# Autodesk Inventor assembly: Lady Brown
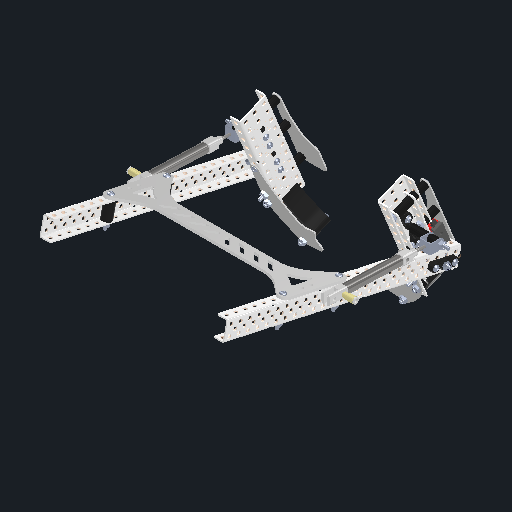
[picture p0: Inventor's stored thumbnail of the model, 512x512]
Saved by Autodesk Inventor 2025.1 (Build 291241000, 241)
## iProperties
Created: 2024-12-19
Part Number: Lady Brown
Document SubType Name: Assembly
Designer: Juan
Author: Juan
## Documents named in this file (36)
- C:\Users\Juanl\Documents\GitHub\ATUM-V5RC-High-Stakes-CAD\Robot\Subassemblies\Lady Brown.iam
- C:\Users\Juanl\Documents\GitHub\ATUM-V5RC-High-Stakes-CAD\VEX-CAD-Inventor\Structure\C Channel\Aluminum 1x2x1\Alu C 1x2x1x25.ipt
- C:\Users\Juanl\Documents\GitHub\ATUM-V5RC-High-Stakes-CAD\VEX-CAD-Inventor\Motion\Spacers\Spacer Nylon .375 OD\NSpacer .375 OD x .500.ipt
- C:\Users\Juan\Documents\GitHub\ATUM-VRC-High-Stakes-CAD\VEX-CAD-Inventor\Motion\Spacers\Spacer Nylon .375 OD.ipt
- C:\Users\Juanl\Documents\GitHub\ATUM-V5RC-High-Stakes-CAD\VEX-CAD-Inventor\Motion\Pneumatics\Reference Parts\Pistons\Double Acting Piston Body.ipt
- C:\Users\Juanl\Documents\GitHub\ATUM-V5RC-High-Stakes-CAD\VEX-CAD-Inventor\Motion\Pneumatics\Reference Parts\Pistons\Double Acting Piston Rod.ipt
- C:\Users\Juanl\Documents\GitHub\ATUM-V5RC-High-Stakes-CAD\VEX-CAD-Inventor\Motion\Pneumatics\Legacy - SMC Pneumatics\Fitting for Cylinders.ipt
- C:\Users\Juanl\Documents\GitHub\ATUM-V5RC-High-Stakes-CAD\VEX-CAD-Inventor\Motion\Shaft LS\Bearing Flat.ipt
- C:\Users\Juanl\Documents\GitHub\ATUM-V5RC-High-Stakes-CAD\VEX-CAD-Inventor\Structure\Hardware\Screw Steel - Star\SScrew Star Smooth .500.ipt
- C:\Users\Juan\Documents\GitHub\ATUM-VRC-High-Stakes-CAD\VEX-CAD-Inventor\Structure\Hardware\Screw Steel - Star.ipt
- C:\Users\Juanl\Documents\GitHub\ATUM-V5RC-High-Stakes-CAD\VEX-CAD-Inventor\Structure\C Channel\Aluminum 1x3x1\Alu C 1x3x1x11.ipt
- C:\Users\Juanl\Documents\GitHub\ATUM-V5RC-High-Stakes-CAD\VEX-CAD-Inventor\Motion\1-Post Bearing Flat Hex Retainer.ipt
- C:\Users\Juanl\Documents\GitHub\ATUM-V5RC-High-Stakes-CAD\VEX-CAD-Inventor\Motion\Pneumatics\Legacy - SMC Pneumatics\Cylinder Mount.ipt
- C:\Users\Juanl\Documents\GitHub\ATUM-V5RC-High-Stakes-CAD\VEX-CAD-Inventor\Motion\Spacers\Spacer Nylon .375 OD\NSpacer .375 OD x .375.ipt
- C:\Users\Juanl\Documents\GitHub\ATUM-V5RC-High-Stakes-CAD\VEX-CAD-Inventor\Structure\Hardware\Screw Steel - Star\SScrew Star Smooth 2.250.ipt
- C:\Users\Juanl\Documents\GitHub\ATUM-V5RC-High-Stakes-CAD\VEX-CAD-Inventor\Structure\Hardware\Nut Nylock.ipt
- C:\Users\Juanl\Documents\GitHub\ATUM-V5RC-High-Stakes-CAD\VEX-CAD-Inventor\Structure\Hardware\Screw Steel - Star\SScrew Star Smooth 1.750.ipt
- C:\Users\Juanl\Documents\GitHub\ATUM-V5RC-High-Stakes-CAD\VEX-CAD-Inventor\Structure\Hardware\Nut Thin Nylock.ipt
- C:\Users\Juanl\Documents\GitHub\ATUM-V5RC-High-Stakes-CAD\VEX-CAD-Inventor\Structure\Hardware\Screw Steel - Star\SScrew Star Smooth .375.ipt
- C:\Users\Juanl\Documents\GitHub\ATUM-V5RC-High-Stakes-CAD\VEX-CAD-Inventor\Motion\Spacers\Spacer Nylon .375 OD\NSpacer .375 OD x .250.ipt
- C:\Users\Juanl\Documents\GitHub\ATUM-V5RC-High-Stakes-CAD\Protobot\Lady Brown Tabs.ipt
- C:\Users\Juanl\Documents\GitHub\ATUM-V5RC-High-Stakes-CAD\Protobot\Lady Brown Tab Top.ipt
- C:\Users\Juanl\Documents\GitHub\ATUM-V5RC-High-Stakes-CAD\VEX-CAD-Inventor\Structure\C Channel\Aluminum 1x2x1\Alu C 1x2x1x8.ipt
- C:\Users\Juanl\Documents\GitHub\ATUM-V5RC-High-Stakes-CAD\VEX-CAD-Inventor\Electronics\Sensors\Line Tracker - V2.ipt
- C:\Users\Juanl\Documents\GitHub\ATUM-V5RC-High-Stakes-CAD\Protobot\Lady Brown Ring Stop.ipt
- C:\Users\Juanl\Documents\GitHub\ATUM-V5RC-High-Stakes-CAD\VEX-CAD-Inventor\Motion\Spacers\Washer Steel\SWasher .375 OD x .062500.ipt
- C:\Users\Juan\Documents\GitHub\ATUM-VRC-High-Stakes-CAD\VEX-CAD-Inventor\Motion\Spacers\Washer Steel.ipt
- C:\Users\Juanl\Documents\GitHub\ATUM-V5RC-High-Stakes-CAD\VEX-CAD-Inventor\Structure\Hardware\Screw Steel - Star\SScrew Star Smooth 1.500.ipt
- C:\Users\Juanl\Documents\GitHub\ATUM-V5RC-High-Stakes-CAD\VEX-CAD-Inventor\Structure\Hardware\Screw Steel - Star\SScrew Star Smooth 2.000.ipt
- C:\Users\Juanl\Documents\GitHub\ATUM-V5RC-High-Stakes-CAD\VEX-CAD-Inventor\Structure\Hardware\Screw Steel - Star\SScrew Star Smooth 2.500.ipt
- C:\Users\Juanl\Documents\GitHub\ATUM-V5RC-High-Stakes-CAD\VEX-CAD-Inventor\Structure\Hardware\Screw Steel - Star\SScrew Star Smooth 1.250.ipt
- C:\Users\Juanl\Documents\GitHub\ATUM-V5RC-High-Stakes-CAD\VEX-CAD-Inventor\Structure\Hardware\Screw Steel - Star\SScrew Star Smooth .625.ipt
- C:\Users\Juanl\Documents\GitHub\ATUM-V5RC-High-Stakes-CAD\Protobot\Lady Brown Arm Brace.ipt
- C:\Users\Juanl\Documents\GitHub\ATUM-V5RC-High-Stakes-CAD\VEX-CAD-Inventor\Motion\Spacers\Spacer Nylon .500 OD\NSpacer Black .500 OD x .500.ipt
- C:\Users\Juan\Documents\GitHub\ATUM-VRC-High-Stakes-CAD\VEX-CAD-Inventor\Motion\Spacers\Spacer Nylon .500 OD.ipt
- C:\Users\Juanl\Documents\GitHub\ATUM-V5RC-High-Stakes-CAD\VEX-CAD-Inventor\Motion\Spacers\Spacer Nylon .500 OD\NSpacer Black .500 OD x .375.ipt
## Components (130 placed, 31 different names)
1. Alu C 1x2x1x25:1 — Mate:103, Mate:104, Mate:105, Rigid:86, Rigid:91, Rigid:98, Rigid:99
2. Alu C 1x2x1x25:2 — Rigid:92, Rigid:93, Rigid:96, Rigid:97
3. Double Acting Piston Body:1
4. Double Acting Piston Rod:1
5. Fitting for Cylinders:1
6. Bearing Flat:1
7. SScrew Star Smooth .500:1
8. SScrew Star Smooth .500:2
9. Alu C 1x3x1x11:1
10. 1-Post Bearing Flat Hex Retainer:1
11. 1-Post Bearing Flat Hex Retainer:2 — Mate:77
12. Cylinder Mount:1
13. NSpacer .375 OD x .375:3 — Mate:78
14. NSpacer .375 OD x .500:4 — Mate:79
15. NSpacer .375 OD x .375:5
16. NSpacer .375 OD x .500:6
17. SScrew Star Smooth 2.250:3
18. Nut Nylock:1
19. SScrew Star Smooth 1.750:4
20. Nut Thin Nylock:1
21. Nut Nylock:2
22. SScrew Star Smooth .375:5
23. SScrew Star Smooth .375:6
24. Nut Nylock:3
25. Double Acting Piston Body:2
26. Double Acting Piston Rod:2
27. NSpacer .375 OD x .500:13
28. NSpacer .375 OD x .375:14
29. Nut Thin Nylock:4
30. Nut Thin Nylock:3
31. Nut Thin Nylock:6
32. Nut Thin Nylock:5
33. SScrew Star Smooth 2.250:12
34. NSpacer .375 OD x .500:12
35. Fitting for Cylinders:2
36. Bearing Flat:2
37. SScrew Star Smooth .500:7
38. SScrew Star Smooth .500:8
39. Alu C 1x3x1x11:2
40. Cylinder Mount:2
41. NSpacer .375 OD x .500:7
42. Nut Nylock:4
43. Nut Thin Nylock:2
44. Nut Nylock:5
45. SScrew Star Smooth .375:9
46. SScrew Star Smooth .375:10
47. Nut Nylock:6
48. 1-Post Bearing Flat Hex Retainer:3 — Mate:93
49. 1-Post Bearing Flat Hex Retainer:4 — Mate:94
50. SScrew Star Smooth 1.750:11
51. NSpacer .375 OD x .500:8 — Mate:95
52. NSpacer .375 OD x .375:9
53. NSpacer .375 OD x .375:15 — Rigid:36, Rigid:41
54. NSpacer .375 OD x .375:16 — Rigid:36, Mate:73, Mate:75, Mate:76
55. NSpacer .375 OD x .250:17 — Mate:70, Mate:72, Rigid:42
56. NSpacer .375 OD x .250:18 — Mate:71, Rigid:43
57. Lady Brown Tabs:2 — Mate:70, Mate:71, Mate:72, Mate:88, Rigid:54, Rigid:56, Rigid:67, Rigid:68, Rigid:78, Rigid:83
58. Lady Brown Tab Top:1 — Mate:73, Mate:75, Mate:76, Mate:83, Rigid:72, Rigid:76, Rigid:79
59. NSpacer .375 OD x .375:21 — Rigid:40
60. NSpacer .375 OD x .375:22 — Mate:83
61. Alu C 1x2x1x8:1 — Mate:77, Mate:78, Mate:79, Rigid:40, Rigid:41, Rigid:42, Rigid:43, Flush:1, Mate:84, Mate:85, Rigid:45, Mate:86, Mate:87, Rigid:71, Rigid:74, Rigid:81, Rigid:84
62. Line Tracker - V2:2 — Flush:1, Mate:84, Mate:85
63. NSpacer .375 OD x .375:23 — Rigid:45
64. NSpacer .375 OD x .375:24
65. Lady Brown Ring Stop:1 — Mate:86, Mate:87, Mate:88, Rigid:62, Rigid:63
66. Lady Brown Ring Stop:2 — Mate:97, Mate:98, Mate:102, Rigid:64, Rotational:3
67. Lady Brown Tabs:3 — Mate:92, Mate:96, Mate:102, Rigid:53, Rigid:55, Rigid:65, Rigid:66, Rigid:77, Rotational:5
68. NSpacer .375 OD x .250:25 — Rigid:46
69. NSpacer .375 OD x .250:26 — Mate:92, Rigid:47, Mate:96
70. Lady Brown Tab Top:2 — Mate:99, Mate:100, Mate:101, Rigid:73, Rigid:75, Rigid:80
71. Alu C 1x2x1x8:2 — Mate:93, Mate:94, Mate:95, Rigid:46, Rigid:47, Mate:97, Mate:98, Mate:99, Mate:100, Rigid:51, Rigid:52, Rotational:2, Rigid:61, Rotational:4, Rigid:82, Rigid:85
72. NSpacer .375 OD x .375:27 — Rigid:51
73. NSpacer .375 OD x .375:28
74. NSpacer .375 OD x .375:29 — Rigid:52
75. NSpacer .375 OD x .375:30 — Mate:101
76. NSpacer .375 OD x .375:31 — Rotational:2
77. NSpacer .375 OD x .375:32
78. NSpacer .375 OD x .250:33 — Rigid:54, Rigid:57
79. NSpacer .375 OD x .250:34 — Rigid:53, Rigid:60
80. NSpacer .375 OD x .250:35 — Rigid:56, Rigid:58
81. NSpacer .375 OD x .250:36 — Rigid:55, Rigid:59
82. SWasher .375 OD x .062500:1 — Rigid:58
83. SWasher .375 OD x .062500:2 — Rigid:57
84. SWasher .375 OD x .062500:3 — Rigid:60
85. SWasher .375 OD x .062500:4 — Rigid:59
86. NSpacer .375 OD x .375:37 — Rigid:61, Rigid:69
87. SScrew Star Smooth 1.500:13 — Rotational:3
88. SScrew Star Smooth 1.500:14 — Rigid:64
89. SScrew Star Smooth 1.500:15 — Rigid:63
90. SScrew Star Smooth 1.500:16 — Rigid:62
91. Nut Thin Nylock:7 — Rigid:65
92. Nut Thin Nylock:8 — Rigid:66
93. Nut Thin Nylock:9 — Rigid:68
94. Nut Thin Nylock:10 — Rigid:67
95. NSpacer .375 OD x .500:38 — Rigid:69
96. NSpacer .375 OD x .375:39 — Rigid:71
97. NSpacer .375 OD x .500:40
98. SScrew Star Smooth 2.000:17 — Rigid:72
99. SScrew Star Smooth 2.000:18 — Rigid:73
100. Nut Thin Nylock:11 — Rigid:74
101. Nut Thin Nylock:12 — Rotational:4
102. SScrew Star Smooth 2.500:20 — Rigid:75
103. SScrew Star Smooth 2.500:21 — Rigid:76
104. Nut Thin Nylock:13 — Rigid:78
105. Nut Thin Nylock:14 — Rigid:77
106. SScrew Star Smooth 1.250:22 — Rigid:80
107. SScrew Star Smooth 1.250:23 — Rigid:79
108. Nut Thin Nylock:15 — Rigid:82
109. Nut Thin Nylock:16 — Rigid:81
110. SScrew Star Smooth .625:24 — Rotational:5
111. SScrew Star Smooth .625:25 — Rigid:83
112. Nut Thin Nylock:17 — Rigid:85
113. Nut Thin Nylock:18 — Rigid:84
114. Lady Brown Arm Brace:1 — Mate:103, Mate:104, Mate:105, Rotational:6, Rigid:94, Rigid:95, Rotational:7
115. NSpacer Black .500 OD x .500:1 — Rigid:86, Rigid:87
116. NSpacer Black .500 OD x .375:2 — Rigid:87
117. NSpacer Black .500 OD x .500:3 — Rigid:91
118. NSpacer Black .500 OD x .375:4
119. NSpacer Black .500 OD x .500:5 — Rigid:93
120. NSpacer Black .500 OD x .375:6
121. NSpacer Black .500 OD x .500:7 — Rigid:92
122. NSpacer Black .500 OD x .375:8
123. SScrew Star Smooth 1.500:26 — Rigid:94
124. SScrew Star Smooth 1.500:27 — Rotational:6
125. SScrew Star Smooth 1.500:28 — Rotational:7
126. SScrew Star Smooth 1.500:29 — Rigid:95
127. Nut Nylock:7 — Rigid:97
128. Nut Nylock:8 — Rigid:96
129. Nut Nylock:9 — Rigid:98
130. Nut Nylock:10 — Rigid:99
## Relationships (177: WeldJoint 94, Mate 73, RevoluteJoint 7, CylindricalJoint 2, Flush 1)
- [Mate]: Double Acting Piston Body:1 ↔ Double Acting Piston Rod:1
- [CylindricalJoint]: Double Acting Piston Body:1 ↔ Double Acting Piston Rod:1
- [Mate]: Double Acting Piston Body:1 ↔ Fitting for Cylinders:1
- [Mate]: Double Acting Piston Body:1 ↔ Fitting for Cylinders:1
- [Mate]: Alu C 1x2x1x25:1 ↔ Bearing Flat:1
- [Mate]: Alu C 1x2x1x25:1 ↔ Bearing Flat:1
- [Mate]: Alu C 1x2x1x25:1 ↔ Bearing Flat:1
- [WeldJoint]: Bearing Flat:1 ↔ SScrew Star Smooth .500:2
- [WeldJoint]: Bearing Flat:1 ↔ SScrew Star Smooth .500:1
- [Mate]: Alu C 1x3x1x11:1 ↔ 1-Post Bearing Flat Hex Retainer:2
- [Mate]: Alu C 1x3x1x11:1 ↔ 1-Post Bearing Flat Hex Retainer:2
- [Mate]: Alu C 1x3x1x11:1 ↔ 1-Post Bearing Flat Hex Retainer:1
- [Mate]: Alu C 1x3x1x11:1 ↔ 1-Post Bearing Flat Hex Retainer:1
- [Mate]: Alu C 1x3x1x11:1 ↔ 1-Post Bearing Flat Hex Retainer:2
- [Mate]: Alu C 1x3x1x11:1 ↔ 1-Post Bearing Flat Hex Retainer:1
- [Mate]: Bearing Flat:1 ↔ 1-Post Bearing Flat Hex Retainer:2
- [Mate]: Double Acting Piston Rod:1 ↔ Cylinder Mount:1
- [Mate]: 1-Post Bearing Flat Hex Retainer:1 ↔ Cylinder Mount:1
- [WeldJoint]: NSpacer .375 OD x .500:4 ↔ NSpacer .375 OD x .375:5
- [Mate]: Cylinder Mount:1 ↔ NSpacer .375 OD x .500:6
- [Mate]: Cylinder Mount:1 ↔ NSpacer .375 OD x .500:6
- [WeldJoint]: Alu C 1x3x1x11:1 ↔ SScrew Star Smooth 2.250:3
- [WeldJoint]: Cylinder Mount:1 ↔ Nut Nylock:1
- [WeldJoint]: Alu C 1x3x1x11:1 ↔ SScrew Star Smooth 1.750:4
- [WeldJoint]: Bearing Flat:1 ↔ Nut Thin Nylock:1
- [WeldJoint]: Alu C 1x3x1x11:1 ↔ SScrew Star Smooth .375:6
- [WeldJoint]: Alu C 1x3x1x11:1 ↔ SScrew Star Smooth .375:5
- [WeldJoint]: 1-Post Bearing Flat Hex Retainer:1 ↔ Nut Nylock:2
- [WeldJoint]: 1-Post Bearing Flat Hex Retainer:2 ↔ Nut Nylock:3
- [Mate]: Double Acting Piston Body:2 ↔ Double Acting Piston Rod:2
- [Mate]: Double Acting Piston Body:2 ↔ Fitting for Cylinders:2
- [Mate]: Double Acting Piston Body:2 ↔ Fitting for Cylinders:2
- [Mate]: Double Acting Piston Rod:2 ↔ Cylinder Mount:2
- [Mate]: Cylinder Mount:2 ↔ NSpacer .375 OD x .500:7
- [CylindricalJoint]: Double Acting Piston Body:2 ↔ Double Acting Piston Rod:2
- [WeldJoint]: Bearing Flat:2 ↔ SScrew Star Smooth .500:7
- [WeldJoint]: Bearing Flat:2 ↔ SScrew Star Smooth .500:8
- [WeldJoint]: Cylinder Mount:2 ↔ Nut Nylock:4
- [WeldJoint]: Bearing Flat:2 ↔ Nut Thin Nylock:2
- [WeldJoint]: Alu C 1x3x1x11:2 ↔ SScrew Star Smooth .375:9
- [WeldJoint]: Alu C 1x3x1x11:2 ↔ SScrew Star Smooth .375:10
- [Mate]: Alu C 1x3x1x11:2 ↔ 1-Post Bearing Flat Hex Retainer:3
- [Mate]: Alu C 1x3x1x11:2 ↔ 1-Post Bearing Flat Hex Retainer:3
- [Mate]: Alu C 1x3x1x11:2 ↔ 1-Post Bearing Flat Hex Retainer:3
- [Mate]: Alu C 1x3x1x11:2 ↔ 1-Post Bearing Flat Hex Retainer:4
- [Mate]: Alu C 1x3x1x11:2 ↔ 1-Post Bearing Flat Hex Retainer:4
- [Mate]: Alu C 1x3x1x11:2 ↔ 1-Post Bearing Flat Hex Retainer:4
- [WeldJoint]: Alu C 1x3x1x11:2 ↔ SScrew Star Smooth 1.750:11
- [Mate]: Alu C 1x2x1x25:2 ↔ Bearing Flat:2
- [Mate]: Alu C 1x2x1x25:2 ↔ Bearing Flat:2
- [Mate]: Alu C 1x2x1x25:2 ↔ Bearing Flat:2
- [Mate]: Bearing Flat:2 ↔ SScrew Star Smooth 1.750:11
- [Mate]: Cylinder Mount:2 ↔ NSpacer .375 OD x .500:7
- [WeldJoint]: Nut Nylock:5 ↔ 1-Post Bearing Flat Hex Retainer:3
- [WeldJoint]: Nut Nylock:6 ↔ 1-Post Bearing Flat Hex Retainer:4
- [WeldJoint]: NSpacer .375 OD x .500:8 ↔ NSpacer .375 OD x .375:9
- [Mate]: Alu C 1x2x1x25:2 ↔ Double Acting Piston Body:2
- [Mate] (0.7937 mm): Alu C 1x2x1x25:2 ↔ Double Acting Piston Body:2
- [Mate]: Alu C 1x3x1x11:1 ↔ Alu C 1x3x1x11:2
- [Mate]: Alu C 1x3x1x11:1 ↔ Alu C 1x3x1x11:2
- [RevoluteJoint] (0.7937 mm): Alu C 1x2x1x25:1 ↔ Double Acting Piston Body:1
- [WeldJoint] (6.35 mm): Double Acting Piston Rod:1 ↔ Cylinder Mount:1
- [WeldJoint] (6.35 mm): Double Acting Piston Rod:2 ↔ Cylinder Mount:2
- [Mate]: Cylinder Mount:2 ↔ NSpacer .375 OD x .375:9
- [Mate]: 1-Post Bearing Flat Hex Retainer:2 ↔ NSpacer .375 OD x .375:3
- [WeldJoint]: Cylinder Mount:1 ↔ NSpacer .375 OD x .375:5
- [WeldJoint]: Alu C 1x2x1x25:1 ↔ NSpacer .375 OD x .500:12
- [WeldJoint]: NSpacer .375 OD x .375:3 ↔ NSpacer .375 OD x .500:12
- [WeldJoint]: NSpacer .375 OD x .500:13 ↔ NSpacer .375 OD x .375:14
- [Mate]: NSpacer .375 OD x .500:13 ↔ SScrew Star Smooth 1.750:11
- [Mate]: Alu C 1x2x1x25:2 ↔ NSpacer .375 OD x .500:13
- [Mate]: NSpacer .375 OD x .375:14 ↔ 1-Post Bearing Flat Hex Retainer:4
- [WeldJoint]: Alu C 1x2x1x25:1 ↔ Nut Thin Nylock:4
- [WeldJoint]: Alu C 1x2x1x25:1 ↔ Nut Thin Nylock:3
- [WeldJoint]: SScrew Star Smooth 2.250:12 ↔ Alu C 1x3x1x11:2
- [WeldJoint]: Alu C 1x2x1x25:2 ↔ Nut Thin Nylock:6
- [WeldJoint]: Alu C 1x2x1x25:2 ↔ Nut Thin Nylock:5
- [Mate]: SScrew Star Smooth 2.250:12 ↔ Nut Nylock:4
- [Mate]: SScrew Star Smooth 2.250:12 ↔ NSpacer .375 OD x .375:9
- Rigid:36 [WeldJoint]: NSpacer .375 OD x .375:15 ↔ NSpacer .375 OD x .375:16
- Mate:70: NSpacer .375 OD x .250:17 ↔ Lady Brown Tabs:2
- Mate:71: NSpacer .375 OD x .250:18 ↔ Lady Brown Tabs:2
- Mate:72: NSpacer .375 OD x .250:17 ↔ Lady Brown Tabs:2
- Mate:73: NSpacer .375 OD x .375:16 ↔ Lady Brown Tab Top:1
- Mate:75: NSpacer .375 OD x .375:16 ↔ Lady Brown Tab Top:1
- Mate:76: NSpacer .375 OD x .375:16 ↔ Lady Brown Tab Top:1
- [WeldJoint]: NSpacer .375 OD x .375:21 ↔ NSpacer .375 OD x .375:22
- Mate:77: 1-Post Bearing Flat Hex Retainer:2 ↔ Alu C 1x2x1x8:1
- Mate:78: NSpacer .375 OD x .375:3 ↔ Alu C 1x2x1x8:1
- Mate:79: NSpacer .375 OD x .500:4 ↔ Alu C 1x2x1x8:1
- Rigid:40 [WeldJoint]: NSpacer .375 OD x .375:21 ↔ Alu C 1x2x1x8:1
- Rigid:41 [WeldJoint]: NSpacer .375 OD x .375:15 ↔ Alu C 1x2x1x8:1
- Rigid:42 [WeldJoint]: NSpacer .375 OD x .250:17 ↔ Alu C 1x2x1x8:1
- Rigid:43 [WeldJoint]: NSpacer .375 OD x .250:18 ↔ Alu C 1x2x1x8:1
- Mate:83: Lady Brown Tab Top:1 ↔ NSpacer .375 OD x .375:22
- Flush:1 (-6.35 mm): Alu C 1x2x1x8:1 ↔ Line Tracker - V2:2
- Mate:84: Alu C 1x2x1x8:1 ↔ Line Tracker - V2:2
- Mate:85: Alu C 1x2x1x8:1 ↔ Line Tracker - V2:2
- [WeldJoint]: NSpacer .375 OD x .375:23 ↔ NSpacer .375 OD x .375:24
- Rigid:45 [WeldJoint]: Alu C 1x2x1x8:1 ↔ NSpacer .375 OD x .375:23
- Mate:86: Alu C 1x2x1x8:1 ↔ Lady Brown Ring Stop:1
- Mate:87: Alu C 1x2x1x8:1 ↔ Lady Brown Ring Stop:1
- Mate:88: Lady Brown Tabs:2 ↔ Lady Brown Ring Stop:1
- Mate:92: Lady Brown Tabs:3 ↔ NSpacer .375 OD x .250:26
- Mate:93: 1-Post Bearing Flat Hex Retainer:3 ↔ Alu C 1x2x1x8:2
- Mate:94: 1-Post Bearing Flat Hex Retainer:4 ↔ Alu C 1x2x1x8:2
- Mate:95: NSpacer .375 OD x .500:8 ↔ Alu C 1x2x1x8:2
- Rigid:46 [WeldJoint]: NSpacer .375 OD x .250:25 ↔ Alu C 1x2x1x8:2
- Rigid:47 [WeldJoint]: NSpacer .375 OD x .250:26 ↔ Alu C 1x2x1x8:2
- Mate:96: Lady Brown Tabs:3 ↔ NSpacer .375 OD x .250:26
- Mate:97: Lady Brown Ring Stop:2 ↔ Alu C 1x2x1x8:2
- Mate:98: Lady Brown Ring Stop:2 ↔ Alu C 1x2x1x8:2
- Mate:99: Lady Brown Tab Top:2 ↔ Alu C 1x2x1x8:2
- Mate:100: Lady Brown Tab Top:2 ↔ Alu C 1x2x1x8:2
- [WeldJoint]: NSpacer .375 OD x .375:27 ↔ NSpacer .375 OD x .375:28
- [WeldJoint]: NSpacer .375 OD x .375:29 ↔ NSpacer .375 OD x .375:30
- [WeldJoint]: NSpacer .375 OD x .375:31 ↔ NSpacer .375 OD x .375:32
- Rigid:51 [WeldJoint]: Alu C 1x2x1x8:2 ↔ NSpacer .375 OD x .375:27
- Rigid:52 [WeldJoint]: Alu C 1x2x1x8:2 ↔ NSpacer .375 OD x .375:29
- Rotational:2 [RevoluteJoint]: Alu C 1x2x1x8:2 ↔ NSpacer .375 OD x .375:31
- Mate:101: Lady Brown Tab Top:2 ↔ NSpacer .375 OD x .375:30
- Mate:102: Lady Brown Ring Stop:2 ↔ Lady Brown Tabs:3
- Rigid:53 [WeldJoint]: Lady Brown Tabs:3 ↔ NSpacer .375 OD x .250:34
- Rigid:54 [WeldJoint]: Lady Brown Tabs:2 ↔ NSpacer .375 OD x .250:33
- Rigid:55 [WeldJoint]: Lady Brown Tabs:3 ↔ NSpacer .375 OD x .250:36
- Rigid:56 [WeldJoint]: Lady Brown Tabs:2 ↔ NSpacer .375 OD x .250:35
- Rigid:57 [WeldJoint]: NSpacer .375 OD x .250:33 ↔ SWasher .375 OD x .062500:2
- Rigid:58 [WeldJoint]: NSpacer .375 OD x .250:35 ↔ SWasher .375 OD x .062500:1
- Rigid:59 [WeldJoint]: NSpacer .375 OD x .250:36 ↔ SWasher .375 OD x .062500:4
- Rigid:60 [WeldJoint]: NSpacer .375 OD x .250:34 ↔ SWasher .375 OD x .062500:3
- Rigid:61 [WeldJoint]: Alu C 1x2x1x8:2 ↔ NSpacer .375 OD x .375:37
- Rigid:62 [WeldJoint]: Lady Brown Ring Stop:1 ↔ SScrew Star Smooth 1.500:16
- Rigid:63 [WeldJoint]: Lady Brown Ring Stop:1 ↔ SScrew Star Smooth 1.500:15
- Rigid:64 [WeldJoint]: Lady Brown Ring Stop:2 ↔ SScrew Star Smooth 1.500:14
- Rotational:3 [RevoluteJoint]: Lady Brown Ring Stop:2 ↔ SScrew Star Smooth 1.500:13
- Rigid:65 [WeldJoint]: Lady Brown Tabs:3 ↔ Nut Thin Nylock:7
- Rigid:66 [WeldJoint]: Lady Brown Tabs:3 ↔ Nut Thin Nylock:8
- Rigid:67 [WeldJoint]: Lady Brown Tabs:2 ↔ Nut Thin Nylock:10
- Rigid:68 [WeldJoint]: Lady Brown Tabs:2 ↔ Nut Thin Nylock:9
- Rigid:69 [WeldJoint]: NSpacer .375 OD x .375:37 ↔ NSpacer .375 OD x .500:38
- [WeldJoint]: NSpacer .375 OD x .375:39 ↔ NSpacer .375 OD x .500:40
- Rigid:71 [WeldJoint]: Alu C 1x2x1x8:1 ↔ NSpacer .375 OD x .375:39
- Rigid:72 [WeldJoint]: Lady Brown Tab Top:1 ↔ SScrew Star Smooth 2.000:17
- Rigid:73 [WeldJoint]: Lady Brown Tab Top:2 ↔ SScrew Star Smooth 2.000:18
- Rigid:74 [WeldJoint]: Alu C 1x2x1x8:1 ↔ Nut Thin Nylock:11
- Rotational:4 [RevoluteJoint]: Alu C 1x2x1x8:2 ↔ Nut Thin Nylock:12
- Rigid:75 [WeldJoint]: Lady Brown Tab Top:2 ↔ SScrew Star Smooth 2.500:20
- Rigid:76 [WeldJoint]: Lady Brown Tab Top:1 ↔ SScrew Star Smooth 2.500:21
- Rigid:77 [WeldJoint]: Lady Brown Tabs:3 ↔ Nut Thin Nylock:14
- Rigid:78 [WeldJoint]: Lady Brown Tabs:2 ↔ Nut Thin Nylock:13
- Rigid:79 [WeldJoint]: Lady Brown Tab Top:1 ↔ SScrew Star Smooth 1.250:23
- Rigid:80 [WeldJoint]: Lady Brown Tab Top:2 ↔ SScrew Star Smooth 1.250:22
- Rigid:81 [WeldJoint]: Alu C 1x2x1x8:1 ↔ Nut Thin Nylock:16
- Rigid:82 [WeldJoint]: Alu C 1x2x1x8:2 ↔ Nut Thin Nylock:15
- Rotational:5 [RevoluteJoint]: Lady Brown Tabs:3 ↔ SScrew Star Smooth .625:24
- Rigid:83 [WeldJoint]: Lady Brown Tabs:2 ↔ SScrew Star Smooth .625:25
- Rigid:84 [WeldJoint]: Alu C 1x2x1x8:1 ↔ Nut Thin Nylock:18
- Rigid:85 [WeldJoint]: Alu C 1x2x1x8:2 ↔ Nut Thin Nylock:17
- Mate:103: Alu C 1x2x1x25:1 ↔ Lady Brown Arm Brace:1
- Mate:104: Alu C 1x2x1x25:1 ↔ Lady Brown Arm Brace:1
- Mate:105: Alu C 1x2x1x25:1 ↔ Lady Brown Arm Brace:1
- Rigid:86 [WeldJoint]: Alu C 1x2x1x25:1 ↔ NSpacer Black .500 OD x .500:1
- Rigid:87 [WeldJoint]: NSpacer Black .500 OD x .500:1 ↔ NSpacer Black .500 OD x .375:2
- [WeldJoint]: NSpacer Black .500 OD x .500:3 ↔ NSpacer Black .500 OD x .375:4
- [WeldJoint]: NSpacer Black .500 OD x .500:5 ↔ NSpacer Black .500 OD x .375:6
- [WeldJoint]: NSpacer Black .500 OD x .500:7 ↔ NSpacer Black .500 OD x .375:8
- Rigid:91 [WeldJoint]: Alu C 1x2x1x25:1 ↔ NSpacer Black .500 OD x .500:3
- Rigid:92 [WeldJoint]: Alu C 1x2x1x25:2 ↔ NSpacer Black .500 OD x .500:7
- Rigid:93 [WeldJoint]: Alu C 1x2x1x25:2 ↔ NSpacer Black .500 OD x .500:5
- Rotational:6 [RevoluteJoint]: Lady Brown Arm Brace:1 ↔ SScrew Star Smooth 1.500:27
- Rigid:94 [WeldJoint]: Lady Brown Arm Brace:1 ↔ SScrew Star Smooth 1.500:26
- Rigid:95 [WeldJoint]: Lady Brown Arm Brace:1 ↔ SScrew Star Smooth 1.500:29
- Rotational:7 [RevoluteJoint]: Lady Brown Arm Brace:1 ↔ SScrew Star Smooth 1.500:28
- Rigid:96 [WeldJoint]: Alu C 1x2x1x25:2 ↔ Nut Nylock:8
- Rigid:97 [WeldJoint]: Alu C 1x2x1x25:2 ↔ Nut Nylock:7
- Rigid:98 [WeldJoint]: Alu C 1x2x1x25:1 ↔ Nut Nylock:9
- Rigid:99 [WeldJoint]: Alu C 1x2x1x25:1 ↔ Nut Nylock:10
## Named parameters: d1821_d1818 = 0 mm, d1789_d1094 = 0 mm, d1790_d1097 = 0 mm, d1791_d1068_d1063 = 0 mm, d1792_d1069_d1064 = 0 deg, d1793_d1070_d1065 = -19.05 mm, d1794_d1071_d1066 = -19.05893 mm, d1795_d1072_d1067 = -69.85 mm, d131_d126_d116 = 0 mm, d152_d116 = 0 mm, d173_d116 = 0 mm, d174_d116 = 0 mm, d175_d116 = 0 mm, d201_d200 = 0 mm, d226_d225 = 0 mm, d227_d225 = 0 mm, d228_d225 = 0 mm
